# Autodesk Inventor assembly: Base Profile-Connector-Plate - Assembly
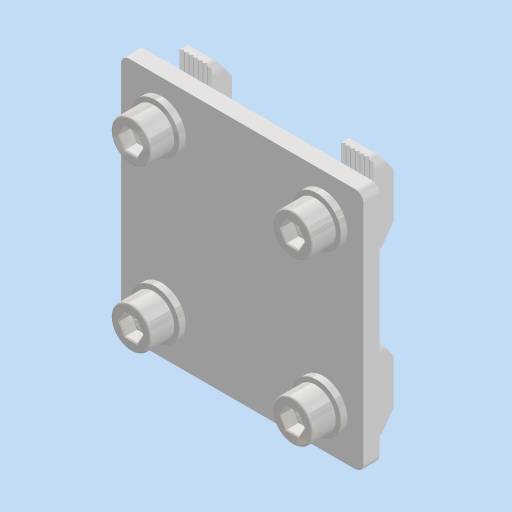
[picture p0: Inventor's stored thumbnail of the model, 512x512]
Saved by Autodesk Inventor 2023.2 (Build 272271000, 271)
## iProperties
Created: 2024-02-21
Part Number: Base Profile-Connector-Plate - Assembly
Document SubType Name: Assembly
Designer: Nils Bade
Author: Nils Bade
## Documents named in this file (6)
- C:\Users\nilsb\Documents\Inventor\Projektarbeit-Bade\RatRig_modified\Base Profile-Connector-Plate - Assembly.iam
- C:\Users\nilsb\Documents\Inventor\Projektarbeit-Bade\RatRig_modified\Base Profile-Connector-Plate.ipt
- C:\Users\nilsb\Documents\Inventor\Projektarbeit-Bade\Schrauben\Cap Head Screw M6x16.ipt
- C:\Users\nilsb\Documents\Inventor\Projektarbeit-Bade\Schrauben\Washer Simple M6 v2.ipt
- Washer Simple M6 1,6mm _DIN125.ipt
- C:\Users\nilsb\Documents\Inventor\Projektarbeit-Bade\RatRig_modified\T-NUT - DropIn 4040 SERIES - M6.ipt
## Components (13 placed, 4 different names)
1. Base Profile-Connector-Plate:1 — Passend:1, Passend:2, Passend:3, Passend:4, Passend:5, Passend:6, Passend:7, Passend:8, Passend:9, Passend:10, Passend:11, Passend:12, Winkel:1, Winkel:2, Winkel:3, Winkel:4, Passend:21, Passend:22, Passend:23, Passend:24
2. Cap Head Screw M6x16:1 — Passend:12, Passend:16, Passend:20
3. Cap Head Screw M6x16:2 — Passend:11, Passend:13, Passend:18
4. Cap Head Screw M6x16:3 — Passend:10, Passend:14, Passend:17
5. Cap Head Screw M6x16:4 — Passend:9, Passend:15, Passend:19
6. Washer Simple M6 1,6mm _DIN125:1 — Passend:4, Passend:8, Passend:16
7. Washer Simple M6 1,6mm _DIN125:2 — Passend:3, Passend:7, Passend:13
8. Washer Simple M6 1,6mm _DIN125:3 — Passend:1, Passend:5, Passend:14
9. Washer Simple M6 1,6mm _DIN125:4 — Passend:2, Passend:6, Passend:15
10. T-NUT - DROP IN TYPE FOR 40 SERIES - M6:1 — Passend:20, Winkel:4, Passend:23
11. T-NUT - DROP IN TYPE FOR 40 SERIES - M6:2 — Passend:19, Winkel:3, Passend:24
12. T-NUT - DROP IN TYPE FOR 40 SERIES - M6:3 — Passend:17, Winkel:2, Passend:22
13. T-NUT - DROP IN TYPE FOR 40 SERIES - M6:4 — Passend:18, Winkel:1, Passend:21
## Relationships (28: Mate 24, Angle 4)
- Passend:1 [Mate]: Base Profile-Connector-Plate:1 ↔ Washer Simple M6 1,6mm _DIN125:3
- Passend:2 [Mate]: Base Profile-Connector-Plate:1 ↔ Washer Simple M6 1,6mm _DIN125:4
- Passend:3 [Mate]: Base Profile-Connector-Plate:1 ↔ Washer Simple M6 1,6mm _DIN125:2
- Passend:4 [Mate]: Base Profile-Connector-Plate:1 ↔ Washer Simple M6 1,6mm _DIN125:1
- Passend:5 [Mate]: Base Profile-Connector-Plate:1 ↔ Washer Simple M6 1,6mm _DIN125:3
- Passend:6 [Mate]: Base Profile-Connector-Plate:1 ↔ Washer Simple M6 1,6mm _DIN125:4
- Passend:7 [Mate]: Base Profile-Connector-Plate:1 ↔ Washer Simple M6 1,6mm _DIN125:2
- Passend:8 [Mate]: Base Profile-Connector-Plate:1 ↔ Washer Simple M6 1,6mm _DIN125:1
- Passend:9 [Mate]: Base Profile-Connector-Plate:1 ↔ Cap Head Screw M6x16:4
- Passend:10 [Mate]: Base Profile-Connector-Plate:1 ↔ Cap Head Screw M6x16:3
- Passend:11 [Mate]: Base Profile-Connector-Plate:1 ↔ Cap Head Screw M6x16:2
- Passend:12 [Mate]: Base Profile-Connector-Plate:1 ↔ Cap Head Screw M6x16:1
- Passend:13 [Mate]: Cap Head Screw M6x16:2 ↔ Washer Simple M6 1,6mm _DIN125:2
- Passend:14 [Mate]: Cap Head Screw M6x16:3 ↔ Washer Simple M6 1,6mm _DIN125:3
- Passend:15 [Mate]: Cap Head Screw M6x16:4 ↔ Washer Simple M6 1,6mm _DIN125:4
- Passend:16 [Mate]: Cap Head Screw M6x16:1 ↔ Washer Simple M6 1,6mm _DIN125:1
- Passend:17 [Mate]: Cap Head Screw M6x16:3 ↔ T-NUT - DROP IN TYPE FOR 40 SERIES - M6:3
- Passend:18 [Mate]: Cap Head Screw M6x16:2 ↔ T-NUT - DROP IN TYPE FOR 40 SERIES - M6:4
- Passend:19 [Mate]: Cap Head Screw M6x16:4 ↔ T-NUT - DROP IN TYPE FOR 40 SERIES - M6:2
- Passend:20 [Mate]: Cap Head Screw M6x16:1 ↔ T-NUT - DROP IN TYPE FOR 40 SERIES - M6:1
- Winkel:1 [Angle] (0 deg): Base Profile-Connector-Plate:1 ↔ T-NUT - DROP IN TYPE FOR 40 SERIES - M6:4
- Winkel:2 [Angle] (0 deg): Base Profile-Connector-Plate:1 ↔ T-NUT - DROP IN TYPE FOR 40 SERIES - M6:3
- Winkel:3 [Angle] (0 deg): Base Profile-Connector-Plate:1 ↔ T-NUT - DROP IN TYPE FOR 40 SERIES - M6:2
- Winkel:4 [Angle] (0 deg): Base Profile-Connector-Plate:1 ↔ T-NUT - DROP IN TYPE FOR 40 SERIES - M6:1
- Passend:21 [Mate] (4.5 mm): Base Profile-Connector-Plate:1 ↔ T-NUT - DROP IN TYPE FOR 40 SERIES - M6:4
- Passend:22 [Mate] (4.5 mm): Base Profile-Connector-Plate:1 ↔ T-NUT - DROP IN TYPE FOR 40 SERIES - M6:3
- Passend:23 [Mate] (4.5 mm): Base Profile-Connector-Plate:1 ↔ T-NUT - DROP IN TYPE FOR 40 SERIES - M6:1
- Passend:24 [Mate] (4.5 mm): Base Profile-Connector-Plate:1 ↔ T-NUT - DROP IN TYPE FOR 40 SERIES - M6:2
